# Autodesk Inventor assembly: ASSEMBLY_Vibration_module
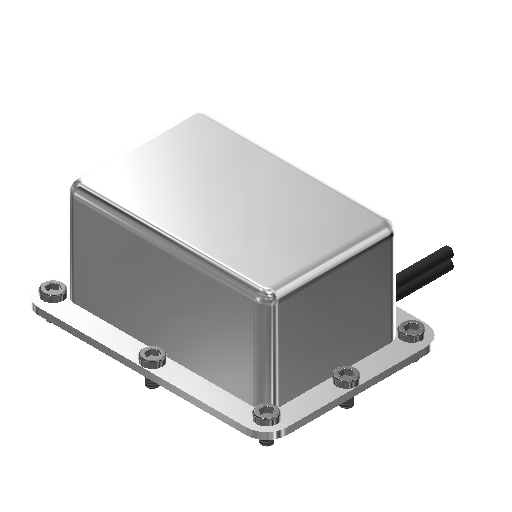
[picture p0: Inventor's stored thumbnail of the model, 512x512]
Saved by Autodesk Inventor 2025 (Build 290162010, 162A)
## iProperties
Created: 2018-09-17
Part Number: ASSEMBLY_Vibration_module
Document SubType Name: Assembly
Designer: Andrzej
Mass: 9.34372 g
Surface Area: 49.6026 cm^2
Volume: 3.28219 cm^3
Density: 2.84679 g/cm^3
Author: Andrzej
## Documents named in this file (3)
- D:\_ANDRZEJ_LACZEWSKI\_OTHER\MECH - My entry for the NASA Lunar Sampling System Design Challenge\MCAD\1_REV1\ASSEMBLY_MAIN_REVA\ASSEMBLY_Vibration_module.iam
- D:\_ANDRZEJ_LACZEWSKI\_OTHER\MECH - My entry for the NASA Lunar Sampling System Design Challenge\MCAD\1_REV1\ASSEMBLY_MAIN_REVA\CNCM_ALU_Vibration_module_cover.ipt
- D:\_ANDRZEJ_LACZEWSKI\_OTHER\MECH - My entry for the NASA Lunar Sampling System Design Challenge\MCAD\1_REV1\ASSEMBLY_MAIN_REVA\CNCT_STEEL_M1,6x3_Screw.ipt
## Components (9 placed, 2 different names)
1. CNCM_ALU_Vibration_module_cover:1 — Mate:1, Mate:2, Mate:3, Mate:4, Mate:5, Mate:6, Mate:7, Mate:8, Mate:9, Mate:10, Mate:11, Mate:12, Mate:13, Mate:14, Mate:15, Mate:16
2. CNCT_STEEL_M1,6x3_Screw:1 — Mate:1, Mate:13
3. CNCT_STEEL_M1,6x3_Screw:2 — Mate:3, Mate:15
4. CNCT_STEEL_M1,6x3_Screw:3 — Mate:5, Mate:10
5. CNCT_STEEL_M1,6x3_Screw:4 — Mate:7, Mate:9
6. CNCT_STEEL_M1,6x3_Screw:5 — Mate:8, Mate:16
7. CNCT_STEEL_M1,6x3_Screw:6 — Mate:6, Mate:12
8. CNCT_STEEL_M1,6x3_Screw:7 — Mate:4, Mate:11
9. CNCT_STEEL_M1,6x3_Screw:8 — Mate:2, Mate:14
## Relationships (16: Mate 16)
- Mate:1: CNCM_ALU_Vibration_module_cover:1 ↔ CNCT_STEEL_M1,6x3_Screw:1
- Mate:2: CNCM_ALU_Vibration_module_cover:1 ↔ CNCT_STEEL_M1,6x3_Screw:8
- Mate:3: CNCM_ALU_Vibration_module_cover:1 ↔ CNCT_STEEL_M1,6x3_Screw:2
- Mate:4: CNCM_ALU_Vibration_module_cover:1 ↔ CNCT_STEEL_M1,6x3_Screw:7
- Mate:5: CNCM_ALU_Vibration_module_cover:1 ↔ CNCT_STEEL_M1,6x3_Screw:3
- Mate:6: CNCM_ALU_Vibration_module_cover:1 ↔ CNCT_STEEL_M1,6x3_Screw:6
- Mate:7: CNCM_ALU_Vibration_module_cover:1 ↔ CNCT_STEEL_M1,6x3_Screw:4
- Mate:8: CNCM_ALU_Vibration_module_cover:1 ↔ CNCT_STEEL_M1,6x3_Screw:5
- Mate:9: CNCM_ALU_Vibration_module_cover:1 ↔ CNCT_STEEL_M1,6x3_Screw:4
- Mate:10: CNCM_ALU_Vibration_module_cover:1 ↔ CNCT_STEEL_M1,6x3_Screw:3
- Mate:11: CNCM_ALU_Vibration_module_cover:1 ↔ CNCT_STEEL_M1,6x3_Screw:7
- Mate:12: CNCM_ALU_Vibration_module_cover:1 ↔ CNCT_STEEL_M1,6x3_Screw:6
- Mate:13: CNCM_ALU_Vibration_module_cover:1 ↔ CNCT_STEEL_M1,6x3_Screw:1
- Mate:14: CNCM_ALU_Vibration_module_cover:1 ↔ CNCT_STEEL_M1,6x3_Screw:8
- Mate:15: CNCM_ALU_Vibration_module_cover:1 ↔ CNCT_STEEL_M1,6x3_Screw:2
- Mate:16: CNCM_ALU_Vibration_module_cover:1 ↔ CNCT_STEEL_M1,6x3_Screw:5
